# Autodesk Inventor assembly: N20Module
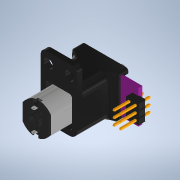
[picture p0: Inventor's stored thumbnail of the model, 180x180]
Saved by Autodesk Inventor 2022 (Build 260153000, 153)
## iProperties
Created: 2021-12-07
Part Number: N20Module
Document SubType Name: Assembly
Designer: JK
Author: JK
## Documents named in this file (6)
- C:\Users\JK\Documents\Inventor\N20 Leg Actuator\N20-Leg-Actuator\CADfiles\N20Module\N20Module.iam
- C:\Users\JK\Documents\Inventor\N20 Leg Actuator\N20-Leg-Actuator\CADfiles\N20Module\Brushed DC Motor v8.iam
- C:\Users\JK\Documents\Inventor\N20 Leg Actuator\N20-Leg-Actuator\CADfiles\N20Module\MotorCase.ipt
- C:\Users\JK\Documents\Inventor\N20 Leg Actuator\N20-Leg-Actuator\CADfiles\N20Module\AngleSensor.ipt
- C:\Users\JK\Documents\Inventor\N20 Leg Actuator\N20-Leg-Actuator\CADfiles\N20Module\adapter.ipt
- C:\Users\JK\Documents\Inventor\N20 Leg Actuator\N20-Leg-Actuator\CADfiles\N20Module\6-Pin Header-Male-Double-2.54mm.ipt
## Components (5 placed, 5 different names)
1. Brushed DC Motor v8:1 [sub-assembly] — Coincidencia:1, Coincidencia:2, Nivelación:1, Coincidencia:4, Ángulo:2
2. MotorCase:1 — Coincidencia:1, Coincidencia:2, Nivelación:1, Coincidencia:3, Ángulo:1
3. AngleSensor:1 — Coincidencia:3, Coincidencia:4, Ángulo:1, Coincidencia:5, Coincidencia:6, Coincidencia:7, Coincidencia:8, Nivelación:2
4. adapter:1 — Coincidencia:5, Ángulo:2, Coincidencia:6
5. 6-Pin Header-Male-Double-2.54mm:1 — Coincidencia:7, Coincidencia:8, Nivelación:2
## Relationships (12: Mate 8, Flush 2, Angle 2)
- Coincidencia:1 [Mate] (0.15 mm): Brushed DC Motor v8:1 ↔ MotorCase:1
- Coincidencia:2 [Mate] (0.15 mm): Brushed DC Motor v8:1 ↔ MotorCase:1
- Nivelación:1 [Flush]: Brushed DC Motor v8:1 ↔ MotorCase:1
- Coincidencia:3 [Mate]: MotorCase:1 ↔ AngleSensor:1
- Coincidencia:4 [Mate]: Brushed DC Motor v8:1 ↔ AngleSensor:1
- Ángulo:1 [Angle] (0 deg): MotorCase:1 ↔ AngleSensor:1
- Coincidencia:5 [Mate]: AngleSensor:1 ↔ adapter:1
- Ángulo:2 [Angle] (0 deg): Brushed DC Motor v8:1 ↔ adapter:1
- Coincidencia:6 [Mate]: AngleSensor:1 ↔ adapter:1
- Coincidencia:7 [Mate] (-2.54 mm): AngleSensor:1 ↔ 6-Pin Header-Male-Double-2.54mm:1
- Coincidencia:8 [Mate]: AngleSensor:1 ↔ 6-Pin Header-Male-Double-2.54mm:1
- Nivelación:2 [Flush] (2.7 mm): AngleSensor:1 ↔ 6-Pin Header-Male-Double-2.54mm:1
